# Autodesk Inventor assembly: BaseMini
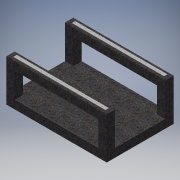
[picture p0: Inventor's stored thumbnail of the model, 180x180]
Saved by Autodesk Inventor 2016 (Build 200138000, 138)
## iProperties
Created: 2015-08-01
Part Number: BaseMini
Document SubType Name: Assembly
Designer: myhome
Mass: 317765 g
Surface Area: 38000 cm^2
Volume: 132000 cm^3
Density: 2.40731 g/cm^3
Author: myhome
## Documents named in this file (4)
- C:\Users\myhome\Documents\Inventor\lasercad\EpoxyGraniteBase\BaseMini.iam
- C:\Users\myhome\Documents\Inventor\lasercad\EpoxyGraniteBase\BaseMini.ipt
- C:\Users\myhome\Documents\Inventor\lasercad\EpoxyGraniteBase\RailsMini.ipt
- C:\Users\myhome\Documents\Inventor\lasercad\FrameSteelPlate\RailBar.ipt
## Components (5 placed, 3 different names)
1. BaseMini:1 — Mate:6, Mate:7, Mate:8, Mate:9, Mate:10, Mate:11
2. RailsMini:1 — Mate:9, Mate:10, Mate:11, Mate:12, Mate:13, Mate:14
3. RailsMini:2 — Mate:6, Mate:7, Mate:8, Mate:15, Mate:16, Mate:17
4. RailBar:1 — Mate:12, Mate:13, Mate:14
5. RailBar:2 — Mate:15, Mate:16, Mate:17
## Relationships (12: Mate 12)
- Mate:6: BaseMini:1 ↔ RailsMini:2
- Mate:7: BaseMini:1 ↔ RailsMini:2
- Mate:8: BaseMini:1 ↔ RailsMini:2
- Mate:9: BaseMini:1 ↔ RailsMini:1
- Mate:10: BaseMini:1 ↔ RailsMini:1
- Mate:11: BaseMini:1 ↔ RailsMini:1
- Mate:12: RailsMini:1 ↔ RailBar:1
- Mate:13: RailsMini:1 ↔ RailBar:1
- Mate:14: RailsMini:1 ↔ RailBar:1
- Mate:15: RailsMini:2 ↔ RailBar:2
- Mate:16: RailsMini:2 ↔ RailBar:2
- Mate:17: RailsMini:2 ↔ RailBar:2
